# Autodesk Inventor assembly: Reductor DerechaSF87_20210618_215747_
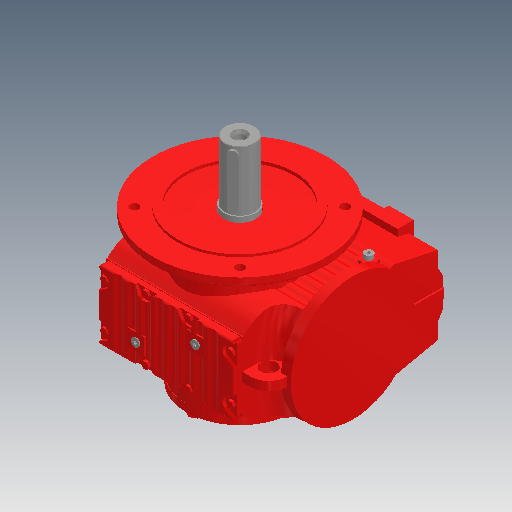
[picture p0: Inventor's stored thumbnail of the model, 512x512]
Saved by Autodesk Inventor 2021 (Build 250183000, 183)
## iProperties
Company: CADClick - www.CADClick.com
Created: 2021-06-18
Part Number: Reductor DerechaSF87_20210618_215747_
Description: STEP AP214
Document SubType Name: Assembly
Designer: Andrés Holguín
Authority: unknown authorization
Preprocessor: Spatial InterOp 3D postprocessed
Title: cctmp_AE05EDE2-B851-4E95-B269-2F44425291F7_2021_6_18_21_57_52_96..stp
Author: SEW-EURODRIVE GmbH & Co KG
Revision Number: NONE
## Documents named in this file (14)
- C:\Users\Santiago Suárez\Documents\GitHub\Dis.-Mecatronico-E6\inventor proyecto\Motores y reductores\Reductor Derecha.iam
- Reductor Derecha.iam
- C:\Users\Santiago Suárez\Documents\GitHub\Dis.-Mecatronico-E6\inventor proyecto\Motores y reductores\Reductor Derecha2021_06_18__21-57-52-065.ipt
- C:\Users\Santiago Suárez\Documents\GitHub\Dis.-Mecatronico-E6\inventor proyecto\Motores y reductores\Reductor Derecha2021_06_18__21-57-52-034.ipt
- C:\Users\Santiago Suárez\Documents\GitHub\Dis.-Mecatronico-E6\inventor proyecto\Motores y reductores\Reductor Derecha2021_06_18__21-57-52-002.ipt
- C:\Users\Santiago Suárez\Documents\GitHub\Dis.-Mecatronico-E6\inventor proyecto\Motores y reductores\Reductor Derecha2021_06_18__21-57-51-971.ipt
- C:\Users\Santiago Suárez\Documents\GitHub\Dis.-Mecatronico-E6\inventor proyecto\Motores y reductores\Reductor Derecha2021_06_18__21-57-51-940.ipt
- C:\Users\Santiago Suárez\Documents\GitHub\Dis.-Mecatronico-E6\inventor proyecto\Motores y reductores\Reductor Derecha2021_06_18__21-57-51-909.ipt
- C:\Users\Santiago Suárez\Documents\GitHub\Dis.-Mecatronico-E6\inventor proyecto\Motores y reductores\Reductor Derecha2021_06_18__21-57-51-877.ipt
- C:\Users\Santiago Suárez\Documents\GitHub\Dis.-Mecatronico-E6\inventor proyecto\Motores y reductores\Reductor Derecha2021_06_18__21-57-51-832.ipt
- C:\Users\Santiago Suárez\Documents\GitHub\Dis.-Mecatronico-E6\inventor proyecto\Motores y reductores\Reductor Derecha2021_06_18__21-57-51-799.ipt
- C:\Users\Santiago Suárez\Documents\GitHub\Dis.-Mecatronico-E6\inventor proyecto\Motores y reductores\Reductor Derecha2021_06_18__21-57-51-768.ipt
- C:\Users\Santiago Suárez\Documents\GitHub\Dis.-Mecatronico-E6\inventor proyecto\Motores y reductores\Reductor Derecha2021_06_18__21-57-51-737.ipt
- C:\Users\Santiago Suárez\Documents\GitHub\Dis.-Mecatronico-E6\inventor proyecto\Motores y reductores\Reductor Derecha2021_06_18__21-57-51-706.ipt
## Components (12 placed, 12 different names)
1. Reductor Derecha2021_06_18__21-57-52-065 — Rotational:3, Rigid:1, Rotational:4, Rigid:2, Rigid:3, Rigid:4, Rotational:5, Rotational:6
2. Reductor Derecha2021_06_18__21-57-52-034 — Rotational:4
3. Reductor Derecha2021_06_18__21-57-52-002 — Rotational:6
4. Reductor Derecha2021_06_18__21-57-51-971 — Rigid:1
5. Reductor Derecha2021_06_18__21-57-51-940 — Rotational:5
6. Reductor Derecha2021_06_18__21-57-51-909 — Rotational:3
7. Reductor Derecha2021_06_18__21-57-51-877 — Rigid:2
8. Reductor Derecha2021_06_18__21-57-51-832 — Rigid:4, Insert:1
9. Reductor Derecha2021_06_18__21-57-51-799 — Insert:1
10. Reductor Derecha2021_06_18__21-57-51-768 — Rotational:1, Rotational:2, Rigid:3
11. Reductor Derecha2021_06_18__21-57-51-737 — Rotational:1
12. Reductor Derecha2021_06_18__21-57-51-706 — Rotational:2
## Relationships (11: RevoluteJoint 6, WeldJoint 4, Insert 1)
- Rotational:1 [RevoluteJoint]: Reductor Derecha2021_06_18__21-57-51-768 ↔ Reductor Derecha2021_06_18__21-57-51-737
- Rotational:2 [RevoluteJoint]: Reductor Derecha2021_06_18__21-57-51-768 ↔ Reductor Derecha2021_06_18__21-57-51-706
- Rotational:3 [RevoluteJoint]: Reductor Derecha2021_06_18__21-57-52-065 ↔ Reductor Derecha2021_06_18__21-57-51-909
- Rigid:1 [WeldJoint]: Reductor Derecha2021_06_18__21-57-52-065 ↔ Reductor Derecha2021_06_18__21-57-51-971
- Rotational:4 [RevoluteJoint]: Reductor Derecha2021_06_18__21-57-52-065 ↔ Reductor Derecha2021_06_18__21-57-52-034
- Rigid:2 [WeldJoint]: Reductor Derecha2021_06_18__21-57-52-065 ↔ Reductor Derecha2021_06_18__21-57-51-877
- Rigid:3 [WeldJoint]: Reductor Derecha2021_06_18__21-57-52-065 ↔ Reductor Derecha2021_06_18__21-57-51-768
- Rigid:4 [WeldJoint]: Reductor Derecha2021_06_18__21-57-52-065 ↔ Reductor Derecha2021_06_18__21-57-51-832
- Insert:1: Reductor Derecha2021_06_18__21-57-51-832 ↔ Reductor Derecha2021_06_18__21-57-51-799
- Rotational:5 [RevoluteJoint]: Reductor Derecha2021_06_18__21-57-52-065 ↔ Reductor Derecha2021_06_18__21-57-51-940
- Rotational:6 [RevoluteJoint]: Reductor Derecha2021_06_18__21-57-52-065 ↔ Reductor Derecha2021_06_18__21-57-52-002
